# Autodesk Inventor assembly: s-assy-unit-magnet
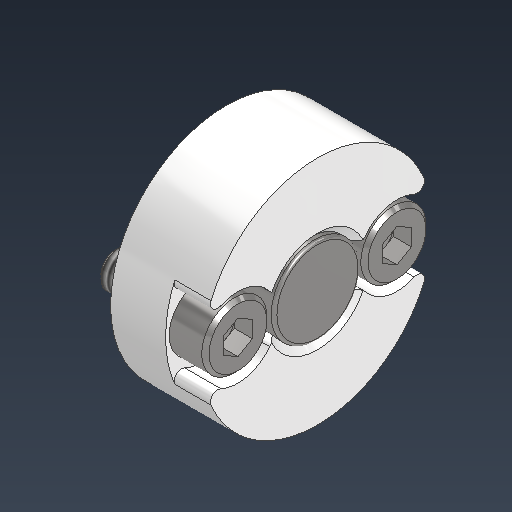
[picture p0: Inventor's stored thumbnail of the model, 512x512]
Saved by Autodesk Inventor 2021 (Build 250183000, 183)
## iProperties
Created: 2021-07-15
Part Number: s-assy-unit-magnet
Document SubType Name: Assembly
Designer: yuta0
Author: yuta0
## Documents named in this file (4)
- C:\Users\yuta0\Documents\GitHub\catchrobo_hardware\assy-robot\s-assy-unit-magnet.iam
- C:\Users\yuta0\Documents\GitHub\catchrobo_hardware\assy-robot\base28.ipt
- C:\Users\yuta0\Documents\GitHub\catchrobo_hardware\assy-robot\magnet.ipt
- C:\Users\yuta0\Documents\GitHub\catchrobo_hardware\assy-robot\CB2_5-6.ipt
## Components (4 placed, 3 different names)
1. base28:1 — メイト:1, メイト:2, メイト:3, メイト:4
2. magnet:1 — メイト:1, メイト:2
3. CB2_5-6:1 — メイト:3, メイト:4
4. CB2_5-6:2
## Component patterns: (2 elements, first: CB2_5-6:1)
## Relationships (4: Mate 4)
- メイト:1 [Mate]: base28:1 ↔ magnet:1
- メイト:2 [Mate]: base28:1 ↔ magnet:1
- メイト:3 [Mate]: base28:1 ↔ CB2_5-6:1
- メイト:4 [Mate]: base28:1 ↔ CB2_5-6:1
